# Autodesk Inventor assembly: złożenie przekładni
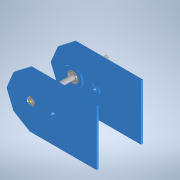
[picture p0: Inventor's stored thumbnail of the model, 180x180]
Saved by Autodesk Inventor 2021 (Build 250183000, 183)
## iProperties
Created: 2021-06-25
Part Number: złożenie przekładni
Document SubType Name: Assembly
Designer: Łukasz
Author: Łukasz
## Documents named in this file (4)
- E:\GITHUB_Czołg\Szybki-Czolg-antyRadziecki\złożenie przekładni.iam
- E:\GITHUB_Czołg\Szybki-Czolg-antyRadziecki\obudowa przekładni.ipt
- C:\Users\Łukasz\Documents\Inventor\Content Center Files\R2021\en-US\BS 292 (I)\BS 292 Part 1 - 608 - 8 x 22 x 7.ipt
- E:\GITHUB_Czołg\Szybki-Czolg-antyRadziecki\oś napędowa.ipt
## Components (4 placed, 3 different names)
1. obudowa przekładni:1 — Rigid:1, Rigid:2
2. BS 292: Part 1 (I) (Metric) 608 - 8 x 22 x 7:2 — Rotational:3, Rigid:2
3. BS 292: Part 1 (I) (Metric) 608 - 8 x 22 x 7:1 — Rigid:1
4. oś napędowa:1 — Rotational:3
## Relationships (3: WeldJoint 2, RevoluteJoint 1)
- Rotational:3 [RevoluteJoint]: BS 292: Part 1 (I) (Metric) 608 - 8 x 22 x 7:2 ↔ oś napędowa:1
- Rigid:1 [WeldJoint]: obudowa przekładni:1 ↔ BS 292: Part 1 (I) (Metric) 608 - 8 x 22 x 7:1
- Rigid:2 [WeldJoint]: obudowa przekładni:1 ↔ BS 292: Part 1 (I) (Metric) 608 - 8 x 22 x 7:2
